# Autodesk Inventor assembly: SAR330 + fixed couplers right
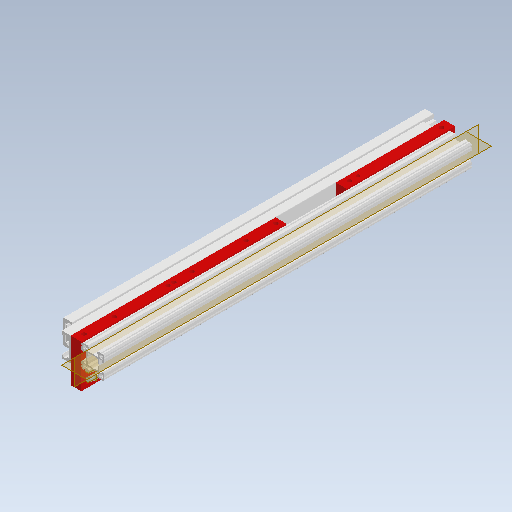
[picture p0: Inventor's stored thumbnail of the model, 512x512]
Saved by Autodesk Inventor 2020 (Build 240168000, 168)
## iProperties
Created: 2019-12-12
Part Number: SAR330 + fixed couplers right
Document SubType Name: Assembly
Designer: ball
Author: ball
## Documents named in this file (7)
- D:\FTC8863\2019 Robot\Delivery\Lift Right\SAR330 + fixed couplers right.iam
- D:\FTC8863\Misumi\SAR330\SAR330 440 offset.iam
- D:\FTC8863\2019 Robot\Delivery\Lift Right\Coupler lift long bottom right + pulleys.iam
- D:\FTC8863\2019 Robot\Delivery\Lift Right\Coupler lift short top right + pulleys.iam
- D:\FTC8863\Actobotics\634 parts\634266.ipt
- D:\FTC8863\Actobotics\565 parts\565046.ipt
- D:\FTC8863\StepLibraries\Screws\M3 x 20 HEX HEAD CAP SCREW.ipt
## Components (6 placed, 6 different names)
1. SAR330 440 offset:1 [sub-assembly] — Mate:1, Mate:2, Mate:3, Mate:4, Mate:5, Flush:1
2. Coupler lift long bottom right + pulleys:1 [sub-assembly] — Mate:1, Mate:2, Mate:3, Mate:6, Mate:7, Mate:8, Flush:2, Flush:3, Mate:9, Mate:10
3. Coupler lift short top right + pulleys:1 [sub-assembly] — Mate:4, Mate:5, Flush:1
4. 634266:1 — Mate:6, Mate:7
5. 565046:1 — Mate:8, Flush:2, Flush:3
6. M3 x 20 HEX HEAD CAP SCREW:1 — Mate:9, Mate:10
## Relationships (13: Mate 10, Flush 3)
- Mate:1: SAR330 440 offset:1 ↔ Coupler lift long bottom right + pulleys:1
- Mate:2: SAR330 440 offset:1 ↔ Coupler lift long bottom right + pulleys:1
- Mate:3: SAR330 440 offset:1 ↔ Coupler lift long bottom right + pulleys:1
- Mate:4: SAR330 440 offset:1 ↔ Coupler lift short top right + pulleys:1
- Mate:5: SAR330 440 offset:1 ↔ Coupler lift short top right + pulleys:1
- Flush:1: SAR330 440 offset:1 ↔ Coupler lift short top right + pulleys:1
- Mate:6: Coupler lift long bottom right + pulleys:1 ↔ 634266:1
- Mate:7: Coupler lift long bottom right + pulleys:1 ↔ 634266:1
- Mate:8: Coupler lift long bottom right + pulleys:1 ↔ 565046:1
- Flush:2: Coupler lift long bottom right + pulleys:1 ↔ 565046:1
- Flush:3: Coupler lift long bottom right + pulleys:1 ↔ 565046:1
- Mate:9: Coupler lift long bottom right + pulleys:1 ↔ M3 x 20 HEX HEAD CAP SCREW:1
- Mate:10: Coupler lift long bottom right + pulleys:1 ↔ M3 x 20 HEX HEAD CAP SCREW:1
